# Autodesk Inventor assembly: Front Right Foot
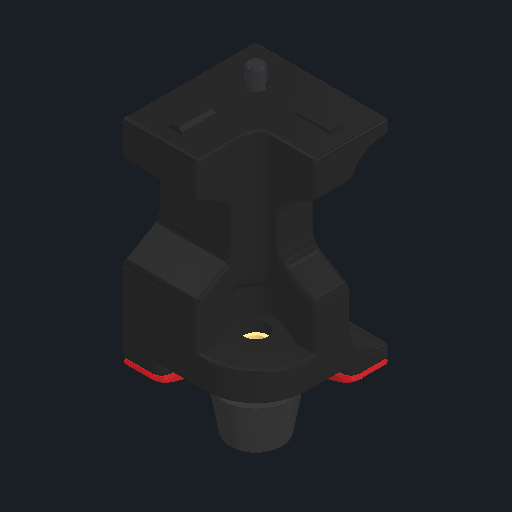
[picture p0: Inventor's stored thumbnail of the model, 512x512]
Saved by Autodesk Inventor 2025.1 (Build 291241020, 241B)
## iProperties
Created: 2025-05-09
Part Number: Front Right Foot
Document SubType Name: Assembly
Designer: AdminForWorker
Title: Front Right Foot
Author: AdminForWorker
## Documents named in this file (7)
- C:\Users\Joshua Eah\Documents\Voron 0.2\CAD\Master Assembly\Front Right Foot.iam
- C:\Users\Joshua Eah\Documents\Voron 0.2\CAD\Master Assembly\Printed Parts (27).iam
- C:\Users\Joshua Eah\Documents\Voron 0.2\CAD\Master Assembly\Hardware\Threaded Insert Assemblies\Threaded Inserts (10).iam
- C:\Users\Joshua Eah\Documents\Voron 0.2\CAD\Master Assembly\Rubber Foot.ipt
- C:\Users\Joshua Eah\Documents\Voron 0.2\CAD\Master Assembly\Hardware\M3x40 BHCS.ipt
- C:\Users\Joshua Eah\Documents\Voron 0.2\CAD\Master Assembly\Hardware\M2x10 Self Tapper.ipt
- C:\Users\Joshua Eah\Documents\Voron 0.2\CAD\Master Assembly\Hardware\M3x10 BHCS.ipt
## Components (7 placed, 6 different names)
1. Printed Parts (27):1 [sub-assembly] — Insert:1, Insert:2
2. Threaded Inserts (10):1 [sub-assembly]
3. Rubber Foot:3
4. M3x40 BHCS:1
5. M2x10 Self Tapper:1 — Insert:1
6. M2x10 Self Tapper:2 — Insert:2
7. M3x10 BHCS:1
## Relationships (2: Insert 2)
- Insert:1: Printed Parts (27):1 ↔ M2x10 Self Tapper:1
- Insert:2: Printed Parts (27):1 ↔ M2x10 Self Tapper:2
